# Autodesk Inventor assembly: 000 ASY GBK Gubkinskiy
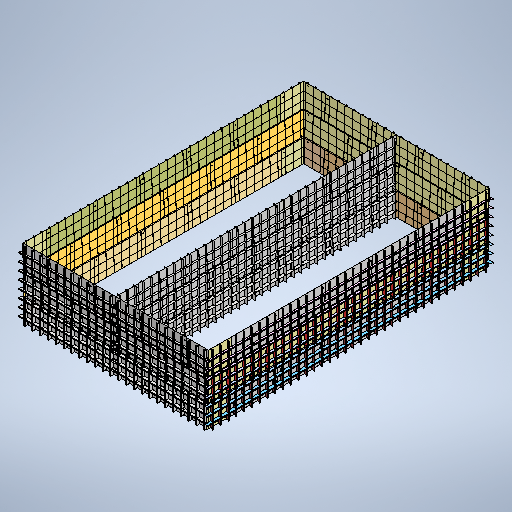
[picture p0: Inventor's stored thumbnail of the model, 512x512]
Saved by Autodesk Inventor 2026.2 (Build 302298010, 298A)
## iProperties
Created: 2026-04-17
Part Number: 000 ASY GBK Gubkinskiy
Document SubType Name: Assembly
Designer: admin
Mass: 2.0116e+07 g
Surface Area: 1.3016e+07 cm^2
Volume: 2.56254e+06 cm^3
Density: 7.85 g/cm^3
Author: admin
## Documents named in this file (6)
- C:\Users\admin\Documents\Inventor\GBK-Gubkinskiy\000 ASY GBK Gubkinskiy.iam
- C:\Users\admin\Documents\Inventor\GBK-Gubkinskiy\GBK bottom.ipt
- C:\Users\admin\Documents\Inventor\GBK-Gubkinskiy\ASY GBK длинная стенка.iam
- C:\Users\admin\Documents\Inventor\GBK-Gubkinskiy\090 ASY bottom.iam
- C:\Users\admin\Documents\Inventor\GBK-Gubkinskiy\ASY GBK короткая стенка.iam
- C:\Users\admin\Documents\Inventor\GBK-Gubkinskiy\ASY GBK центральная стенка.iam
## Components (7 placed, 5 different names)
1. GBK bottom.ipt:1 — Flush:8, Flush:9, Mate:20, Mate:21, Flush:14, Flush:15, Mate:22, Flush:16, Mate:23, Flush:19, Flush:20, Flush:21, Flush:22, Mate:24, Mate:25, Mate:26
2. ASY GBK длинная стенка.iam:1 [sub-assembly] — Flush:15, Flush:20
3. ASY GBK длинная стенка.iam:2 [sub-assembly] — Flush:9, Mate:21, Flush:14
4. 090 ASY bottom.iam:1 [sub-assembly] — Mate:19, Flush:8
5. ASY GBK короткая стенка.iam:1 [sub-assembly] — Mate:20, Flush:19, Mate:25, Mate:27
6. ASY GBK короткая стенка.iam:2 [sub-assembly] — Mate:22, Flush:16, Mate:26
7. ASY GBK центральная стенка.iam:1 [sub-assembly] — Mate:23, Flush:18, Mate:27
## Relationships (20: Mate 10, Flush 10)
- [Mate]: GBK bottom.ipt:1 ↔ ASY GBK длинная стенка.iam:1
- Mate:19: 090 ASY bottom.iam:1
- Flush:8: GBK bottom.ipt:1 ↔ 090 ASY bottom.iam:1
- Flush:9 (-120 mm): GBK bottom.ipt:1 ↔ ASY GBK длинная стенка.iam:2
- Mate:20: GBK bottom.ipt:1 ↔ ASY GBK короткая стенка.iam:1
- Mate:21: GBK bottom.ipt:1 ↔ ASY GBK длинная стенка.iam:2
- Flush:14 (40 mm): GBK bottom.ipt:1 ↔ ASY GBK длинная стенка.iam:2
- Flush:15 (40 mm): GBK bottom.ipt:1 ↔ ASY GBK длинная стенка.iam:1
- Mate:22: GBK bottom.ipt:1 ↔ ASY GBK короткая стенка.iam:2
- Flush:16 (40 mm): GBK bottom.ipt:1 ↔ ASY GBK короткая стенка.iam:2
- Mate:23: GBK bottom.ipt:1 ↔ ASY GBK центральная стенка.iam:1
- Flush:18 (-2 mm): ASY GBK центральная стенка.iam:1
- Flush:19 (40 mm): GBK bottom.ipt:1 ↔ ASY GBK короткая стенка.iam:1
- Flush:20 (120 mm): GBK bottom.ipt:1 ↔ ASY GBK длинная стенка.iam:1
- Flush:21: GBK bottom.ipt:1
- Flush:22: GBK bottom.ipt:1
- Mate:24: GBK bottom.ipt:1
- Mate:25 (-360 mm): GBK bottom.ipt:1 ↔ ASY GBK короткая стенка.iam:1
- Mate:26 (-360 mm): GBK bottom.ipt:1 ↔ ASY GBK короткая стенка.iam:2
- Mate:27 (1.254 mm): ASY GBK короткая стенка.iam:1 ↔ ASY GBK центральная стенка.iam:1
## Named parameters: Зазор_по_горизонту = 1 mm, d120_Зазор_по_горизонту = 1 mm, d141_Зазор_по_горизонту = 1 mm, d159_d141_Зазор_по_горизонту = 1 mm, d175_d141_Зазор_по_горизонту = 1 mm
